# Autodesk Inventor assembly: gears
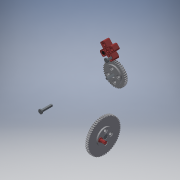
[picture p0: Inventor's stored thumbnail of the model, 180x180]
Saved by Autodesk Inventor 2019 (Build 230136000, 136)
## iProperties
Created: 2019-01-24
Part Number: gears
Document SubType Name: Assembly
Designer: Varga Daniel
Author: Varga Daniel
## Documents named in this file (6)
- C:\!_Dani\!_cloud\OneDrive\!_munka\Revolution\RevvyDemoKit\Structural parts\Demo parts\Gears\gears.iam
- C:\!_Dani\!_cloud\OneDrive\!_munka\Revolution\RevvyDemoKit\Structural parts\Connetor Pins\cp1x1.ipt
- C:\!_Dani\!_cloud\OneDrive\!_munka\Revolution\RevvyDemoKit\Structural parts\Axle Connectors\Axle connector 3x3 cross.ipt
- C:\!_Dani\!_cloud\OneDrive\!_munka\Revolution\RevvyDemoKit\Structural parts\Demo parts\Gears\gear40.iam
- C:\!_Dani\!_cloud\OneDrive\!_munka\Revolution\RevvyDemoKit\Structural parts\Axles\Axle 2.ipt
- C:\!_Dani\!_cloud\OneDrive\!_munka\Revolution\RevvyDemoKit\Structural parts\Demo parts\Gears\gear60.iam
## Components (9 placed, 5 different names)
1. cp1x1:1 — Mate:3, Mate:4
2. gear40:1 [sub-assembly] — Mate:5, Mate:6, Angle:1
3. Axle connector 3x3 cross:2 — Mate:3, Mate:4, Mate:7
4. Axle 2:1 — Mate:5, Mate:6, Angle:1
5. Axle 2:2 — Mate:7
6. gear60:1 [sub-assembly] — Mate:8, Mate:9, Mate:10, Mate:11
7. Axle 2:3
8. Axle 2:4 — Mate:8, Mate:9
9. cp1x1:2 — Mate:10, Mate:11
## Relationships (10: Mate 9, Angle 1)
- Mate:3: cp1x1:1 ↔ Axle connector 3x3 cross:2
- Mate:4: cp1x1:1 ↔ Axle connector 3x3 cross:2
- Mate:5: gear40:1 ↔ Axle 2:1
- Mate:6: gear40:1 ↔ Axle 2:1
- Angle:1 (0 deg): gear40:1 ↔ Axle 2:1
- Mate:7: Axle connector 3x3 cross:2 ↔ Axle 2:2
- Mate:8: gear60:1 ↔ Axle 2:4
- Mate:9: gear60:1 ↔ Axle 2:4
- Mate:10: gear60:1 ↔ cp1x1:2
- Mate:11: gear60:1 ↔ cp1x1:2
